# Autodesk Inventor assembly: 5-10
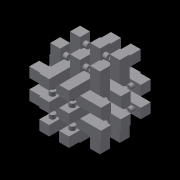
[picture p0: Inventor's stored thumbnail of the model, 180x180]
Saved by Autodesk Inventor 2017 (Build 210142000, 142)
## iProperties
Part Number: 5-10
Material: 一般
Document SubType Name: Assembly
Designer: r0909
Author: r0909
## Documents named in this file (3)
- C:\Users\r0909\Desktop\inventor\5-10.iam
- C:\Users\r0909\Desktop\inventor\5-8.ipt
- C:\Users\r0909\Desktop\inventor\5-9.ipt
## Components (18 placed, 2 different names)
1. 5-8:1 — 齊平:1, 齊平:2, 貼合:1, 齊平:3, 齊平:4, 齊平:5, 貼合:2, 貼合:6, 相切:1
2. 5-9:1 — 齊平:17, 齊平:18, 貼合:12, 貼合:13, 貼合:17, 相切:10
3. 5-8:2 — 齊平:1, 齊平:2, 貼合:1, 齊平:6, 貼合:3, 相切:2
4. 5-8:3 — 齊平:3, 齊平:5, 貼合:2, 齊平:7, 齊平:8, 貼合:4, 貼合:9, 貼合:10, 相切:3
5. 5-8:4 — 齊平:4, 齊平:6, 貼合:3, 齊平:9, 齊平:10, 貼合:5, 相切:4
6. 5-8:5 — 齊平:9, 齊平:10, 貼合:5, 貼合:14, 貼合:15, 貼合:18, 貼合:19, 相切:7, 相切:8
7. 5-8:6 — 齊平:7, 齊平:8, 貼合:4, 相切:5, 相切:6, 貼合:21, 相切:9, 貼合:23, 相切:11
8. 5-8:7 — 貼合:6, 相切:1, 相切:2, 齊平:11, 齊平:12, 貼合:7
9. 5-8:8 — 齊平:11, 齊平:12, 貼合:7, 齊平:13, 齊平:14, 貼合:8
10. 5-8:9 — 齊平:13, 齊平:14, 貼合:8, 齊平:15
11. 5-8:10 — 齊平:15, 齊平:16, 貼合:9, 貼合:11, 相切:3, 相切:4, 貼合:16, 貼合:20
12. 5-8:11 — 齊平:16, 貼合:10, 貼合:11, 齊平:17, 齊平:18, 貼合:12, 貼合:22, 貼合:24
13. 5-8:12 — 貼合:13, 相切:5, 貼合:14
14. 5-8:13 — 貼合:15, 貼合:16, 相切:6
15. 5-8:14 — 貼合:17, 貼合:18, 相切:8
16. 5-8:15 — 貼合:19, 貼合:20, 相切:7
17. 5-8:16 — 貼合:21, 貼合:22, 相切:9, 相切:10
18. 5-8:17 — 貼合:23, 貼合:24, 相切:11
## Relationships (53: Mate 24, Flush 18, Tangent 11)
- 齊平:1 [Flush]: 5-8:1 ↔ 5-8:2
- 齊平:2 [Flush]: 5-8:1 ↔ 5-8:2
- 貼合:1 [Mate] (9 mm): 5-8:1 ↔ 5-8:2
- 齊平:3 [Flush]: 5-8:1 ↔ 5-8:3
- 齊平:4 [Flush]: 5-8:1 ↔ 5-8:4
- 齊平:5 [Flush]: 5-8:1 ↔ 5-8:3
- 齊平:6 [Flush]: 5-8:2 ↔ 5-8:4
- 貼合:2 [Mate] (9 mm): 5-8:1 ↔ 5-8:3
- 貼合:3 [Mate] (9 mm): 5-8:2 ↔ 5-8:4
- 齊平:7 [Flush]: 5-8:3 ↔ 5-8:6
- 齊平:8 [Flush]: 5-8:3 ↔ 5-8:6
- 齊平:9 [Flush]: 5-8:4 ↔ 5-8:5
- 齊平:10 [Flush]: 5-8:4 ↔ 5-8:5
- 貼合:4 [Mate] (9 mm): 5-8:3 ↔ 5-8:6
- 貼合:5 [Mate] (9 mm): 5-8:4 ↔ 5-8:5
- 貼合:6 [Mate]: 5-8:1 ↔ 5-8:7
- 相切:1 [Tangent]: 5-8:1 ↔ 5-8:7
- 相切:2 [Tangent]: 5-8:2 ↔ 5-8:7
- 齊平:11 [Flush]: 5-8:7 ↔ 5-8:8
- 齊平:12 [Flush]: 5-8:7 ↔ 5-8:8
- 貼合:7 [Mate] (9 mm): 5-8:7 ↔ 5-8:8
- 齊平:13 [Flush]: 5-8:8 ↔ 5-8:9
- 齊平:14 [Flush]: 5-8:8 ↔ 5-8:9
- 貼合:8 [Mate] (9 mm): 5-8:8 ↔ 5-8:9
- 齊平:15 [Flush]: 5-8:9 ↔ 5-8:10
- 齊平:16 [Flush]: 5-8:10 ↔ 5-8:11
- 貼合:9 [Mate]: 5-8:3 ↔ 5-8:10
- 貼合:10 [Mate]: 5-8:3 ↔ 5-8:11
- 貼合:11 [Mate] (9 mm): 5-8:10 ↔ 5-8:11
- 相切:3 [Tangent]: 5-8:3 ↔ 5-8:10
- 相切:4 [Tangent]: 5-8:4 ↔ 5-8:10
- 齊平:17 [Flush]: 5-9:1 ↔ 5-8:11
- 齊平:18 [Flush]: 5-9:1 ↔ 5-8:11
- 貼合:12 [Mate] (9 mm): 5-9:1 ↔ 5-8:11
- 貼合:13 [Mate]: 5-9:1 ↔ 5-8:12
- 相切:5 [Tangent]: 5-8:6 ↔ 5-8:12
- 貼合:14 [Mate]: 5-8:5 ↔ 5-8:12
- 貼合:15 [Mate]: 5-8:5 ↔ 5-8:13
- 貼合:16 [Mate]: 5-8:10 ↔ 5-8:13
- 相切:6 [Tangent]: 5-8:6 ↔ 5-8:13
- 貼合:17 [Mate]: 5-9:1 ↔ 5-8:14
- 貼合:18 [Mate]: 5-8:5 ↔ 5-8:14
- 貼合:19 [Mate]: 5-8:5 ↔ 5-8:15
- 貼合:20 [Mate]: 5-8:10 ↔ 5-8:15
- 相切:7 [Tangent]: 5-8:5 ↔ 5-8:15
- 相切:8 [Tangent]: 5-8:5 ↔ 5-8:14
- 貼合:21 [Mate]: 5-8:6 ↔ 5-8:16
- 貼合:22 [Mate]: 5-8:11 ↔ 5-8:16
- 相切:9 [Tangent]: 5-8:6 ↔ 5-8:16
- 相切:10 [Tangent]: 5-9:1 ↔ 5-8:16
- 貼合:23 [Mate]: 5-8:6 ↔ 5-8:17
- 貼合:24 [Mate]: 5-8:11 ↔ 5-8:17
- 相切:11 [Tangent]: 5-8:6 ↔ 5-8:17
